# Autodesk Inventor assembly: Arm 2.0 Assembly
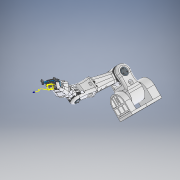
[picture p0: Inventor's stored thumbnail of the model, 180x180]
Saved by Autodesk Inventor 2017 SP1 (Build 210196100, 196)
## iProperties
Created: 2017-09-28
Part Number: Arm 2.0 Assembly
Document SubType Name: Assembly
Designer: Zach
Author: Zach
## Documents named in this file (46)
- C:\Users\Zach\Documents\GitHub\tr1\src\Body\Arm 2.0 Assembly\Arm 2.0 Assembly.iam
- C:\Users\Zach\Documents\GitHub\tr1\src\Body\Arm 2.0 Assembly\Steel Rod 8mm x 135mm.ipt
- C:\Users\Zach\Documents\GitHub\tr1\lib\22x8x8mm Bearing.ipt
- C:\Users\Zach\Documents\GitHub\tr1\src\Body\Arm 2.0 Assembly\AA004.ipt
- C:\Users\Zach\Documents\GitHub\tr1\src\Body\Arm 2.0 Assembly\AA005.ipt
- C:\Users\Zach\Documents\GitHub\tr1\src\Body\Arm 2.0 Assembly\AA006.ipt
- C:\Users\Zach\Documents\GitHub\tr1\src\Body\Arm 2.0 Assembly\AA007.ipt
- C:\Users\Zach\Documents\GitHub\tr1\lib\QS12MM250\QS12MM250.ipt
- C:\Users\Zach\Documents\GitHub\tr1\src\Body\Arm 2.0 Assembly\AA008.ipt
- C:\Users\Zach\Documents\GitHub\tr1\lib\13x4x5mm Bearing.ipt
- C:\Users\Zach\Documents\GitHub\tr1\src\Body\Arm 2.0 Assembly\AA010.ipt
- C:\Users\Zach\Documents\GitHub\tr1\src\Body\Arm 2.0 Assembly\AA011.ipt
- C:\Users\Zach\Documents\GitHub\tr1\src\Body\Arm 2.0 Assembly\AA012.ipt
- C:\Users\Zach\Documents\GitHub\tr1\src\Body\Arm 2.0 Assembly\Steel Rod 8mm x 100mm.ipt
- C:\Users\Zach\Documents\GitHub\tr1\src\Body\Arm 2.0 Assembly\AA013.ipt
- C:\Users\Zach\Documents\GitHub\tr1\src\Body\Arm 2.0 Assembly\AA014.ipt
- C:\Users\Zach\Documents\GitHub\tr1\src\Body\Arm 2.0 Assembly\AA016.ipt
- C:\Users\Zach\Documents\GitHub\tr1\src\Body\Arm 2.0 Assembly\AA017.ipt
- C:\Users\Zach\Documents\GitHub\tr1\lib\12V DC Motor 378-1.ipt
- C:\Users\Zach\Documents\Inventor\Content Center Files\R2017\en-US\ISO 4016\ISO 4016 - M5 x 25.ipt
- C:\Users\Zach\Documents\Inventor\Content Center Files\R2017\en-US\ISO 4017(1)\ISO 4017 - M5 x 12 - ISO.ipt
- C:\Users\Zach\Documents\Inventor\Content Center Files\R2017\en-US\ISO 4017(1)\ISO 4017 - M5 x 20 - ISO.ipt
- C:\Users\Zach\Documents\GitHub\tr1\src\Body\Arm 2.0 Assembly\AA019.ipt
- C:\Users\Zach\Documents\GitHub\tr1\src\Body\Arm 2.0 Assembly\AA020.ipt
- C:\Users\Zach\Documents\GitHub\tr1\src\Body\Arm 2.0 Assembly\AA021.ipt
- C:\Users\Zach\Documents\GitHub\tr1\src\Body\Arm 2.0 Assembly\AA022.ipt
- C:\Users\Zach\Documents\GitHub\tr1\src\Body\Arm 2.0 Assembly\Steel Rod 8mm x 80mm.ipt
- C:\Users\Zach\Documents\GitHub\tr1\src\Body\Arm 2.0 Assembly\AA023.ipt
- C:\Users\Zach\Documents\GitHub\BCN3D-Moveo\Autodesk Inventor files\Gripper B Assembly.iam
- C:\Users\Zach\Documents\Inventor\Content Center Files\R2017\en-US\CNS 4320\CNS 4320 - M8 x 1 x 100.ipt
- C:\Users\Zach\Documents\GitHub\tr1\src\Body\Arm 2.0 Assembly\AA027.ipt
- C:\Users\Zach\Documents\GitHub\tr1\lib\AS 1110 - M8 x 150.ipt
- C:\Users\Zach\Documents\GitHub\tr1\src\Body\Arm 2.0 Assembly\AA029.ipt
- C:\Users\Zach\Documents\GitHub\tr1\src\Body\Arm 2.0 Assembly\AA030.ipt
- C:\Users\Zach\Documents\GitHub\tr1\lib\8mm Hub.ipt
- C:\Users\Zach\Documents\GitHub\tr1\src\Body\Arm 2.0 Assembly\Arm 2.0 Assembly\Design Accelerator\Spur Gears5.iam
- C:\Users\Zach\Documents\GitHub\tr1\lib\4mm mounting hub.ipt
- C:\Users\Zach\Documents\GitHub\tr1\lib\6201RS\6201RS.ipt
- C:\Users\Zach\Documents\GitHub\tr1\lib\U51105\U51105.ipt
- C:\Users\Zach\Documents\GitHub\tr1\src\Body\Arm 2.0 Assembly\AA033.ipt
- C:\Users\Zach\Documents\GitHub\tr1\src\Body\Arm 2.0 Assembly\AA032.ipt
- C:\Users\Zach\Documents\GitHub\tr1\src\Body\Arm 2.0 Assembly\AA031.ipt
- C:\Users\Zach\Documents\GitHub\tr1\lib\Timing Pulley - T5 4mm Bore 15mm Width.ipt
- C:\Users\Zach\Documents\GitHub\tr1\src\Body\Arm 2.0 Assembly\AA034.ipt
- C:\Users\Zach\Documents\GitHub\tr1\src\Body\Arm 2.0 Assembly\Arm 2.0 Assembly\Design Accelerator\Spur Gears6.iam
- C:\Users\Zach\Documents\GitHub\tr1\src\Body\Arm 2.0 Assembly\AA001b.ipt
## Components (89 placed, 44 different names)
1. AA001b:1 — Mate:414, Mate:415, Mate:416, Mate:421, Mate:422, Mate:423, Mate:431, Mate:432, Flush:18, Flush:19, Mate:434, Mate:435, Flush:20, Mate:438, Mate:439, Mate:440, Mate:443, Mate:444, Mate:445
2. AA004:1 — Mate:12, Mate:13, Mate:15, Mate:23, Mate:345, Mate:347, Mate:350, Mate:352, Mate:353, Mate:357, Mate:414, Mate:431, Mate:435
3. AA005:1 — Mate:99, Mate:100, Mate:103, Mate:331, Mate:332, Mate:333, Mate:341, Mate:381
4. AA006:1 — Mate:24, Mate:25, Mate:96, Mate:97, Mate:98, Mate:382, Mate:383
5. AA007:1 — Mate:19, Mate:20, Mate:99, Mate:100, Mate:103
6. AA007:2 — Mate:19, Mate:20, Mate:96, Mate:97, Mate:98
7. AA008:1 — Mate:35, Mate:36, Mate:39, Mate:41, Mate:43, Mate:46, Mate:276, Mate:277, Mate:278, Mate:279, Mate:280, Mate:281, Mate:282, Mate:293, Mate:309, Mate:428, Mate:429, Mate:430, Mate:441
8. AA010:1 — Mate:52, Mate:53, Mate:55, Flush:6, Mate:56, Flush:7, Flush:8, Mate:64, Mate:65, Mate:66, Mate:67, Mate:68, Mate:69, Mate:107, Mate:108, Mate:109, Mate:317, Mate:318, Mate:319, Mate:330, Mate:377, Mate:402, Mate:403, Mate:404, Mate:405, Mate:406, Mate:407
9. AA011:1 — Mate:49, Mate:50, Mate:51, Flush:9, Mate:79, Mate:81, Mate:273
10. AA012:1 — Mate:49, Mate:50, Mate:51, Mate:52, Mate:53, Flush:9, Mate:80
11. AA013:1 — Mate:148, Mate:149, Mate:150, Mate:151, Mate:152, Mate:153, Mate:434, Mate:436
12. AA013:2 — Mate:142, Mate:143, Mate:144, Mate:145, Mate:146, Mate:147, Mate:439
13. AA014:1 — Mate:64, Mate:65, Mate:66, Mate:160, Mate:161, Mate:162, Mate:163, Mate:164, Mate:165
14. AA014:2 — Mate:67, Mate:68, Mate:69, Mate:154, Mate:155, Mate:156, Mate:157, Mate:158, Mate:159
15. AA016:1 — Mate:79, Mate:80, Mate:81, Mate:245, Mate:246, Mate:247, Mate:260, Mate:261, Mate:262, Mate:263, Mate:274, Mate:364, Mate:442
16. AA017:2 — Mate:403, Mate:404, Mate:407
17. AA017:3 — Mate:402, Mate:405, Mate:406
18. AA019:1 — Mate:174, Mate:175, Mate:182, Mate:183, Mate:185, Flush:15, Flush:16, Flush:17, Mate:188, Mate:189, Mate:190, Mate:191, Mate:192, Mate:193, Mate:387, Mate:388, Mate:389, Mate:390, Mate:400, Mate:401
19. AA020:1 — Mate:171, Mate:172, Mate:173, Mate:175, Mate:194, Mate:196
20. AA021:1 — Mate:171, Mate:172, Mate:173, Mate:174, Mate:195
21. AA022:3 — Mate:384, Mate:389, Mate:390, Mate:391, Mate:442
22. AA023:1 — Mate:188, Mate:189, Mate:193
23. AA023:2 — Mate:190, Mate:191, Mate:192
24. AA027:1 — Mate:273, Mate:274
25. AA029:1 — Mate:309, Mate:311, Mate:312, Mate:313, Mate:314, Mate:315, Mate:316, Mate:323, Mate:359, Mate:441
26. AA030:1 — Mate:317, Mate:318, Mate:319, Mate:322, Mate:323
27. AA031:1 — Mate:365, Mate:366, Mate:367
28. AA032:1 — Mate:360, Mate:361, Mate:362, Mate:408
29. AA033:1 — Mate:351, Mate:352, Mate:353, Mate:355, Mate:356
30. AA034:1 — Mate:384, Mate:385, Mate:386, Mate:387, Mate:388, Mate:391
31. Gripper B Assembly:1 [sub-assembly] — Mate:194, Mate:195, Mate:196
32. 13x4x5mm Bearing:1 — Mate:35, Mate:36
33. 13x4x5mm Bearing:2 — Mate:313, Mate:314
34. 13x4x5mm Bearing:3 — Mate:315, Mate:316
35. 13x4x5mm Bearing:4 — Mate:39, Mate:43
36. 13x4x5mm Bearing:5 — Mate:311, Mate:312
37. 13x4x5mm Bearing:6 — Mate:41, Mate:46
38. 22x8x8mm Bearing:1 — Mate:433, Flush:18
39. 22x8x8mm Bearing:2 — Mate:437, Flush:20
40. 22x8x8mm Bearing:3 — Mate:55, Flush:6, Mate:57
41. 22x8x8mm Bearing:4 — Mate:56, Flush:7
42. 22x8x8mm Bearing:5 — Mate:186, Flush:16
43. 22x8x8mm Bearing:6 — Mate:187, Flush:17
44. 22x8x8mm Bearing:7 — Mate:262, Mate:263, Mate:264
45. 22x8x8mm Bearing:8 — Mate:260, Mate:261
46. 22x8x8mm Bearing:11 — Mate:281, Mate:282
47. 22x8x8mm Bearing:12 — Mate:279, Mate:280
48. QS12MM250:1 — Mate:23, Mate:24, Mate:25, Mate:344, Mate:346, Mate:348, Mate:351, Mate:354
49. Steel Rod 8mm x 135mm:1 — Mate:432, Mate:433, Flush:19, Mate:436, Mate:437, Mate:448
50. Steel Rod 8mm x 100mm:1 — Mate:57, Flush:8
51. Steel Rod 8mm x 80mm:1 — Mate:185, Flush:15, Mate:186, Mate:187
52. 12V DC Motor 378-1:1 — Mate:371, Mate:421, Mate:422, Mate:423, Mate:446
53. 12V DC Motor 378-1:2 — Mate:107, Mate:108, Mate:109, Mate:376, Mate:378
54. 12V DC Motor 378-1:3 — Mate:182, Mate:183, Mate:392, Mate:394, Mate:400
55. 12V DC Motor 378-1:4 — Mate:245, Mate:246, Mate:247, Mate:363, Mate:365
56. 12V DC Motor 378-1:5 — Mate:276, Mate:277, Mate:278, Mate:358, Mate:360
57. 12V DC Motor 378-1:6 — Mate:331, Mate:332, Mate:333, Mate:340, Mate:342
58. 6201RS:1 — Mate:346, Mate:347
59. 6201RS:2 — Mate:356, Mate:357
60. U51105:1 — Mate:348, Mate:349, Mate:381
61. U51105:2 — Mate:354, Mate:355, Mate:382, Mate:383
62. 8mm Hub:1 — Mate:329, Mate:330
63. 8mm Hub:2 — Mate:368, Mate:386
64. 4mm mounting hub:1 — Mate:340, Mate:341, Mate:343
65. 4mm mounting hub:2 — Mate:358, Mate:359, Mate:361, Mate:362
66. 4mm mounting hub:3 — Mate:363, Mate:364, Mate:366, Mate:367
67. 4mm mounting hub:4 — Mate:371, Mate:443
68. 4mm mounting hub:5 — Mate:376, Mate:377, Mate:397
69. 4mm mounting hub:6 — Mate:392, Mate:395, Mate:396, Mate:401
70. Timing Pulley - T5 4mm Bore 15mm Width:2 — Mate:378, Mate:397
71. Timing Pulley - T5 4mm Bore 15mm Width:3 — Mate:394, Mate:395, Mate:396
72. ISO 4016 M5 x 25:9 — Mate:415
73. ISO 4016 M5 x 25:10 — Mate:416
74. ISO 4017 M5 x 20:1 — Mate:146, Mate:147, Mate:438
75. ISO 4017 M5 x 20:2 — Mate:144, Mate:145, Mate:440
76. ISO 4017 M5 x 20:3 — Mate:142, Mate:143
77. ISO 4017 M5 x 20:4 — Mate:148, Mate:149
78. ISO 4017 M5 x 20:5 — Mate:152, Mate:153
79. ISO 4017 M5 x 20:6 — Mate:150, Mate:151
80. ISO 4017 M5 x 12:1 — Mate:154, Mate:155
81. ISO 4017 M5 x 12:2 — Mate:156, Mate:158
82. ISO 4017 M5 x 12:3 — Mate:157, Mate:159
83. ISO 4017 M5 x 12:4 — Mate:160, Mate:161
84. ISO 4017 M5 x 12:5 — Mate:162, Mate:163
85. ISO 4017 M5 x 12:6 — Mate:164, Mate:165
86. CNS 4320 M8 x 100:1 — Mate:264, Mate:368, Mate:385
87. AS 1110 - Metric M8 x 80:1 — Mate:293, Mate:322, Mate:329, Mate:408
88. Spur Gears:5 [sub-assembly] — Mate:342, Mate:343, Mate:344, Mate:345, Mate:349, Mate:350
89. Spur Gears:6 [sub-assembly] — Mate:428, Mate:429, Mate:430, Mate:444, Mate:445, Mate:446, Mate:448
## Relationships (212: Mate 202, Flush 10)
- Mate:12: AA004:1
- Mate:13: AA004:1
- Mate:15: AA004:1
- Mate:19: AA007:1 ↔ AA007:2
- Mate:20: AA007:1 ↔ AA007:2
- Mate:23: AA004:1 ↔ QS12MM250:1
- Mate:24: AA006:1 ↔ QS12MM250:1
- Mate:25: AA006:1 ↔ QS12MM250:1
- Mate:35: AA008:1 ↔ 13x4x5mm Bearing:1
- Mate:36: AA008:1 ↔ 13x4x5mm Bearing:1
- Mate:39: AA008:1 ↔ 13x4x5mm Bearing:4
- Mate:41: AA008:1 ↔ 13x4x5mm Bearing:6
- Mate:43: AA008:1 ↔ 13x4x5mm Bearing:4
- Mate:46: AA008:1 ↔ 13x4x5mm Bearing:6
- Mate:49: AA011:1 ↔ AA012:1
- Mate:50: AA011:1 ↔ AA012:1
- Mate:51: AA011:1 ↔ AA012:1
- Mate:52: AA010:1 ↔ AA012:1
- Mate:53 (1.75 mm): AA010:1 ↔ AA012:1
- Mate:55: AA010:1 ↔ 22x8x8mm Bearing:3
- Flush:6: AA010:1 ↔ 22x8x8mm Bearing:3
- Mate:56: AA010:1 ↔ 22x8x8mm Bearing:4
- Flush:7: AA010:1 ↔ 22x8x8mm Bearing:4
- Mate:57: 22x8x8mm Bearing:3 ↔ Steel Rod 8mm x 100mm:1
- Flush:8 (2.5 mm): AA010:1 ↔ Steel Rod 8mm x 100mm:1
- Mate:64: AA010:1 ↔ AA014:1
- Mate:65: AA010:1 ↔ AA014:1
- Mate:66: AA010:1 ↔ AA014:1
- Mate:67: AA010:1 ↔ AA014:2
- Mate:68: AA010:1 ↔ AA014:2
- Mate:69: AA010:1 ↔ AA014:2
- Flush:9: AA011:1 ↔ AA012:1
- Mate:79: AA011:1 ↔ AA016:1
- Mate:80: AA012:1 ↔ AA016:1
- Mate:81: AA011:1 ↔ AA016:1
- Mate:96: AA006:1 ↔ AA007:2
- Mate:97: AA006:1 ↔ AA007:2
- Mate:98: AA006:1 ↔ AA007:2
- Mate:99: AA005:1 ↔ AA007:1
- Mate:100: AA005:1 ↔ AA007:1
- Mate:103: AA005:1 ↔ AA007:1
- Mate:107: AA010:1 ↔ 12V DC Motor 378-1:2
- Mate:108: AA010:1 ↔ 12V DC Motor 378-1:2
- Mate:109: AA010:1 ↔ 12V DC Motor 378-1:2
- Mate:142: AA013:2 ↔ ISO 4017 M5 x 20:3
- Mate:143: AA013:2 ↔ ISO 4017 M5 x 20:3
- Mate:144: AA013:2 ↔ ISO 4017 M5 x 20:2
- Mate:145: AA013:2 ↔ ISO 4017 M5 x 20:2
- Mate:146: AA013:2 ↔ ISO 4017 M5 x 20:1
- Mate:147: AA013:2 ↔ ISO 4017 M5 x 20:1
- Mate:148: AA013:1 ↔ ISO 4017 M5 x 20:4
- Mate:149: AA013:1 ↔ ISO 4017 M5 x 20:4
- Mate:150: AA013:1 ↔ ISO 4017 M5 x 20:6
- Mate:151: AA013:1 ↔ ISO 4017 M5 x 20:6
- Mate:152: AA013:1 ↔ ISO 4017 M5 x 20:5
- Mate:153: AA013:1 ↔ ISO 4017 M5 x 20:5
- Mate:154: AA014:2 ↔ ISO 4017 M5 x 12:1
- Mate:155: AA014:2 ↔ ISO 4017 M5 x 12:1
- Mate:156: AA014:2 ↔ ISO 4017 M5 x 12:2
- Mate:157: AA014:2 ↔ ISO 4017 M5 x 12:3
- Mate:158: AA014:2 ↔ ISO 4017 M5 x 12:2
- Mate:159: AA014:2 ↔ ISO 4017 M5 x 12:3
- Mate:160: AA014:1 ↔ ISO 4017 M5 x 12:4
- Mate:161: AA014:1 ↔ ISO 4017 M5 x 12:4
- Mate:162: AA014:1 ↔ ISO 4017 M5 x 12:5
- Mate:163: AA014:1 ↔ ISO 4017 M5 x 12:5
- Mate:164: AA014:1 ↔ ISO 4017 M5 x 12:6
- Mate:165: AA014:1 ↔ ISO 4017 M5 x 12:6
- Mate:171: AA020:1 ↔ AA021:1
- Mate:172: AA020:1 ↔ AA021:1
- Mate:173: AA020:1 ↔ AA021:1
- Mate:174 (1 mm): AA019:1 ↔ AA021:1
- Mate:175: AA019:1 ↔ AA020:1
- Mate:182: AA019:1 ↔ 12V DC Motor 378-1:3
- Mate:183: AA019:1 ↔ 12V DC Motor 378-1:3
- Mate:185: AA019:1 ↔ Steel Rod 8mm x 80mm:1
- Flush:15: AA019:1 ↔ Steel Rod 8mm x 80mm:1
- Mate:186: 22x8x8mm Bearing:5 ↔ Steel Rod 8mm x 80mm:1
- Flush:16: AA019:1 ↔ 22x8x8mm Bearing:5
- Mate:187: 22x8x8mm Bearing:6 ↔ Steel Rod 8mm x 80mm:1
- Flush:17: AA019:1 ↔ 22x8x8mm Bearing:6
- Mate:188: AA019:1 ↔ AA023:1
- Mate:189: AA019:1 ↔ AA023:1
- Mate:190: AA019:1 ↔ AA023:2
- Mate:191: AA019:1 ↔ AA023:2
- Mate:192: AA019:1 ↔ AA023:2
- Mate:193: AA019:1 ↔ AA023:1
- Mate:194: AA020:1 ↔ Gripper B Assembly:1
- Mate:195: AA021:1 ↔ Gripper B Assembly:1
- Mate:196: AA020:1 ↔ Gripper B Assembly:1
- Mate:245: AA016:1 ↔ 12V DC Motor 378-1:4
- Mate:246: AA016:1 ↔ 12V DC Motor 378-1:4
- Mate:247: AA016:1 ↔ 12V DC Motor 378-1:4
- Mate:260: AA016:1 ↔ 22x8x8mm Bearing:8
- Mate:261 (0.5 mm): AA016:1 ↔ 22x8x8mm Bearing:8
- Mate:262: AA016:1 ↔ 22x8x8mm Bearing:7
- Mate:263 (0.5 mm): AA016:1 ↔ 22x8x8mm Bearing:7
- Mate:264: 22x8x8mm Bearing:7 ↔ CNS 4320 M8 x 100:1
- Mate:273: AA011:1 ↔ AA027:1
- Mate:274: AA016:1 ↔ AA027:1
- Mate:276: AA008:1 ↔ 12V DC Motor 378-1:5
- Mate:277: AA008:1 ↔ 12V DC Motor 378-1:5
- Mate:278: AA008:1 ↔ 12V DC Motor 378-1:5
- Mate:279: AA008:1 ↔ 22x8x8mm Bearing:12
- Mate:280 (0.5 mm): AA008:1 ↔ 22x8x8mm Bearing:12
- Mate:281: AA008:1 ↔ 22x8x8mm Bearing:11
- Mate:282 (0.5 mm): AA008:1 ↔ 22x8x8mm Bearing:11
- Mate:293: AA008:1 ↔ AS 1110 - Metric M8 x 80:1
- Mate:309: AA008:1 ↔ AA029:1
- Mate:311: AA029:1 ↔ 13x4x5mm Bearing:5
- Mate:312: AA029:1 ↔ 13x4x5mm Bearing:5
- Mate:313: AA029:1 ↔ 13x4x5mm Bearing:2
- Mate:314: AA029:1 ↔ 13x4x5mm Bearing:2
- Mate:315: AA029:1 ↔ 13x4x5mm Bearing:3
- Mate:316: AA029:1 ↔ 13x4x5mm Bearing:3
- Mate:317: AA010:1 ↔ AA030:1
- Mate:318: AA010:1 ↔ AA030:1
- Mate:319: AA010:1 ↔ AA030:1
- Mate:322: AA030:1 ↔ AS 1110 - Metric M8 x 80:1
- Mate:323 (2.5 mm): AA029:1 ↔ AA030:1
- Mate:329: 8mm Hub:1 ↔ AS 1110 - Metric M8 x 80:1
- Mate:330: AA010:1 ↔ 8mm Hub:1
- Mate:331: AA005:1 ↔ 12V DC Motor 378-1:6
- Mate:332: AA005:1 ↔ 12V DC Motor 378-1:6
- Mate:333: AA005:1 ↔ 12V DC Motor 378-1:6
- Mate:340: 12V DC Motor 378-1:6 ↔ 4mm mounting hub:1
- Mate:341: AA005:1 ↔ 4mm mounting hub:1
- Mate:342: 12V DC Motor 378-1:6 ↔ Spur Gears:5
- Mate:343: 4mm mounting hub:1 ↔ Spur Gears:5
- Mate:344: QS12MM250:1 ↔ Spur Gears:5
- Mate:345: AA004:1 ↔ Spur Gears:5
- Mate:346: QS12MM250:1 ↔ 6201RS:1
- Mate:347: AA004:1 ↔ 6201RS:1
- Mate:348: QS12MM250:1 ↔ U51105:1
- Mate:349: U51105:1 ↔ Spur Gears:5
- Mate:350: AA004:1 ↔ Spur Gears:5
- Mate:351: AA033:1 ↔ QS12MM250:1
- Mate:352: AA004:1 ↔ AA033:1
- Mate:353: AA004:1 ↔ AA033:1
- Mate:354: QS12MM250:1 ↔ U51105:2
- Mate:355: AA033:1 ↔ U51105:2
- Mate:356: AA033:1 ↔ 6201RS:2
- Mate:357: AA004:1 ↔ 6201RS:2
- Mate:358: 12V DC Motor 378-1:5 ↔ 4mm mounting hub:2
- Mate:359: AA029:1 ↔ 4mm mounting hub:2
- Mate:360: AA032:1 ↔ 12V DC Motor 378-1:5
- Mate:361: AA032:1 ↔ 4mm mounting hub:2
- Mate:362: AA032:1 ↔ 4mm mounting hub:2
- Mate:363: 12V DC Motor 378-1:4 ↔ 4mm mounting hub:3
- Mate:364: AA016:1 ↔ 4mm mounting hub:3
- Mate:365: AA031:1 ↔ 12V DC Motor 378-1:4
- Mate:366: AA031:1 ↔ 4mm mounting hub:3
- Mate:367: AA031:1 ↔ 4mm mounting hub:3
- Mate:368: 8mm Hub:2 ↔ CNS 4320 M8 x 100:1
- Mate:371: 12V DC Motor 378-1:1 ↔ 4mm mounting hub:4
- Mate:376: 12V DC Motor 378-1:2 ↔ 4mm mounting hub:5
- Mate:377: AA010:1 ↔ 4mm mounting hub:5
- Mate:378: 12V DC Motor 378-1:2 ↔ Timing Pulley - T5 4mm Bore 15mm Width:2
- Mate:381 (1 mm): AA005:1 ↔ U51105:1
- Mate:382: AA006:1 ↔ U51105:2
- Mate:383: AA006:1 ↔ U51105:2
- Mate:384: AA022:3 ↔ AA034:1
- Mate:385: AA034:1 ↔ CNS 4320 M8 x 100:1
- Mate:386: AA034:1 ↔ 8mm Hub:2
- Mate:387: AA019:1 ↔ AA034:1
- Mate:388: AA019:1 ↔ AA034:1
- Mate:389: AA019:1 ↔ AA022:3
- Mate:390: AA019:1 ↔ AA022:3
- Mate:391: AA022:3 ↔ AA034:1
- Mate:392: 12V DC Motor 378-1:3 ↔ 4mm mounting hub:6
- Mate:394: 12V DC Motor 378-1:3 ↔ Timing Pulley - T5 4mm Bore 15mm Width:3
- Mate:395: 4mm mounting hub:6 ↔ Timing Pulley - T5 4mm Bore 15mm Width:3
- Mate:396: 4mm mounting hub:6 ↔ Timing Pulley - T5 4mm Bore 15mm Width:3
- Mate:397: 4mm mounting hub:5 ↔ Timing Pulley - T5 4mm Bore 15mm Width:2
- Mate:400: AA019:1 ↔ 12V DC Motor 378-1:3
- Mate:401: AA019:1 ↔ 4mm mounting hub:6
- Mate:402: AA010:1 ↔ AA017:3
- Mate:403: AA010:1 ↔ AA017:2
- Mate:404: AA010:1 ↔ AA017:2
- Mate:405: AA010:1 ↔ AA017:3
- Mate:406: AA010:1 ↔ AA017:3
- Mate:407: AA010:1 ↔ AA017:2
- Mate:408: AA032:1 ↔ AS 1110 - Metric M8 x 80:1
- Mate:414: AA001b:1 ↔ AA004:1
- Mate:415: AA001b:1 ↔ ISO 4016 M5 x 25:9
- Mate:416: AA001b:1 ↔ ISO 4016 M5 x 25:10
- Mate:421: AA001b:1 ↔ 12V DC Motor 378-1:1
- Mate:422: AA001b:1 ↔ 12V DC Motor 378-1:1
- Mate:423: AA001b:1 ↔ 12V DC Motor 378-1:1
- Mate:428: AA008:1 ↔ Spur Gears:6
- Mate:429: AA008:1 ↔ Spur Gears:6
- Mate:430: AA008:1 ↔ Spur Gears:6
- Mate:431: AA001b:1 ↔ AA004:1
- Mate:432: AA001b:1 ↔ Steel Rod 8mm x 135mm:1
- Mate:433: 22x8x8mm Bearing:1 ↔ Steel Rod 8mm x 135mm:1
- Flush:18: AA001b:1 ↔ 22x8x8mm Bearing:1
- Flush:19 (-2.5 mm): AA001b:1 ↔ Steel Rod 8mm x 135mm:1
- Mate:434: AA001b:1 ↔ AA013:1
- Mate:435: AA001b:1 ↔ AA004:1
- Mate:436: AA013:1 ↔ Steel Rod 8mm x 135mm:1
- Mate:437: 22x8x8mm Bearing:2 ↔ Steel Rod 8mm x 135mm:1
- Flush:20: AA001b:1 ↔ 22x8x8mm Bearing:2
- Mate:438: AA001b:1 ↔ ISO 4017 M5 x 20:1
- Mate:439: AA001b:1 ↔ AA013:2
- Mate:440: AA001b:1 ↔ ISO 4017 M5 x 20:2
- Mate:441: AA008:1 ↔ AA029:1
- Mate:442 (2.5 mm): AA016:1 ↔ AA022:3
- Mate:443 (1.625 mm): AA001b:1 ↔ 4mm mounting hub:4
- Mate:444 (1.625 mm): AA001b:1 ↔ Spur Gears:6
- Mate:445 (1.625 mm): AA001b:1 ↔ Spur Gears:6
- Mate:446: 12V DC Motor 378-1:1 ↔ Spur Gears:6
- Mate:448: Steel Rod 8mm x 135mm:1 ↔ Spur Gears:6
